# Autodesk Inventor assembly: S8x1
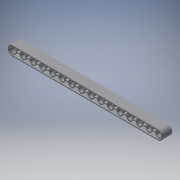
[picture p0: Inventor's stored thumbnail of the model, 180x180]
Saved by Autodesk Inventor 2019 (Build 230136000, 136)
## iProperties
Created: 2019-01-31
Part Number: S8x1
Document SubType Name: Assembly
Designer: Varga Daniel
Author: Varga Daniel
## Documents named in this file (3)
- C:\!_Dani\!_cloud\OneDrive\!_munka\Revolution\RevvyDemoKit\Structural parts\Straight Beams\S16x1.iam
- C:\!_Dani\!_cloud\OneDrive\!_munka\Revolution\RevvyDemoKit\Structural parts\Straight Beams\straight_beam_inner_part_single.ipt
- C:\!_Dani\!_cloud\OneDrive\!_munka\Revolution\RevvyDemoKit\Structural parts\Straight Beams\straight_beam_end_part_single.ipt
## Components (16 placed, 2 different names)
1. straight_beam_inner_part_single:1 — Mate:4, Mate:5, Flush:25, Flush:26, Flush:27, Flush:28, Flush:29, Flush:30
2. straight_beam_inner_part_single:2 — Mate:5, Flush:11, Flush:12, Mate:7, Flush:25, Flush:26
3. straight_beam_inner_part_single:3 — Mate:3, Mate:4, Flush:29, Flush:30
4. straight_beam_inner_part_single:4 — Mate:2, Mate:3, Flush:27, Flush:28, Flush:31, Flush:32
5. straight_beam_inner_part_single:5 — Mate:2, Flush:23, Flush:24, Flush:31, Flush:32, Mate:13
6. straight_beam_end_part_single:1 — Flush:41, Flush:42, Mate:18
7. straight_beam_end_part_single:2 — Flush:11, Flush:12, Mate:7
8. straight_beam_inner_part_single:6 — Flush:13, Flush:14, Mate:8, Flush:15, Flush:16, Mate:9
9. straight_beam_inner_part_single:7 — Flush:15, Flush:16, Mate:9, Flush:17, Flush:18, Mate:10
10. straight_beam_inner_part_single:8 — Flush:17, Flush:18, Mate:10, Flush:19, Flush:20, Mate:11
11. straight_beam_inner_part_single:9 — Flush:19, Flush:20, Mate:11, Flush:33, Flush:34, Mate:14
12. straight_beam_inner_part_single:10 — Flush:13, Flush:14, Mate:8, Flush:23, Flush:24, Mate:13
13. straight_beam_inner_part_single:11 — Flush:33, Flush:34, Flush:35, Flush:36, Mate:14, Mate:15
14. straight_beam_inner_part_single:12 — Flush:35, Flush:36, Flush:37, Flush:38, Mate:15, Mate:16
15. straight_beam_inner_part_single:13 — Flush:37, Flush:38, Flush:39, Flush:40, Mate:16, Mate:17
16. straight_beam_inner_part_single:14 — Flush:39, Flush:40, Flush:41, Flush:42, Mate:17, Mate:18
## Relationships (45: Flush 30, Mate 15)
- Mate:2: straight_beam_inner_part_single:4 ↔ straight_beam_inner_part_single:5
- Mate:3: straight_beam_inner_part_single:3 ↔ straight_beam_inner_part_single:4
- Mate:4: straight_beam_inner_part_single:1 ↔ straight_beam_inner_part_single:3
- Mate:5: straight_beam_inner_part_single:1 ↔ straight_beam_inner_part_single:2
- Flush:11: straight_beam_inner_part_single:2 ↔ straight_beam_end_part_single:2
- Flush:12: straight_beam_inner_part_single:2 ↔ straight_beam_end_part_single:2
- Mate:7: straight_beam_inner_part_single:2 ↔ straight_beam_end_part_single:2
- Flush:13: straight_beam_inner_part_single:6 ↔ straight_beam_inner_part_single:10
- Flush:14: straight_beam_inner_part_single:6 ↔ straight_beam_inner_part_single:10
- Mate:8: straight_beam_inner_part_single:6 ↔ straight_beam_inner_part_single:10
- Flush:15: straight_beam_inner_part_single:6 ↔ straight_beam_inner_part_single:7
- Flush:16: straight_beam_inner_part_single:6 ↔ straight_beam_inner_part_single:7
- Mate:9: straight_beam_inner_part_single:6 ↔ straight_beam_inner_part_single:7
- Flush:17: straight_beam_inner_part_single:7 ↔ straight_beam_inner_part_single:8
- Flush:18: straight_beam_inner_part_single:7 ↔ straight_beam_inner_part_single:8
- Mate:10: straight_beam_inner_part_single:7 ↔ straight_beam_inner_part_single:8
- Flush:19: straight_beam_inner_part_single:8 ↔ straight_beam_inner_part_single:9
- Flush:20: straight_beam_inner_part_single:8 ↔ straight_beam_inner_part_single:9
- Mate:11: straight_beam_inner_part_single:8 ↔ straight_beam_inner_part_single:9
- Flush:23: straight_beam_inner_part_single:5 ↔ straight_beam_inner_part_single:10
- Flush:24: straight_beam_inner_part_single:5 ↔ straight_beam_inner_part_single:10
- Flush:25: straight_beam_inner_part_single:1 ↔ straight_beam_inner_part_single:2
- Flush:26: straight_beam_inner_part_single:1 ↔ straight_beam_inner_part_single:2
- Flush:27: straight_beam_inner_part_single:1 ↔ straight_beam_inner_part_single:4
- Flush:28: straight_beam_inner_part_single:1 ↔ straight_beam_inner_part_single:4
- Flush:29: straight_beam_inner_part_single:1 ↔ straight_beam_inner_part_single:3
- Flush:30: straight_beam_inner_part_single:1 ↔ straight_beam_inner_part_single:3
- Flush:31: straight_beam_inner_part_single:4 ↔ straight_beam_inner_part_single:5
- Flush:32: straight_beam_inner_part_single:4 ↔ straight_beam_inner_part_single:5
- Mate:13: straight_beam_inner_part_single:5 ↔ straight_beam_inner_part_single:10
- Flush:33: straight_beam_inner_part_single:9 ↔ straight_beam_inner_part_single:11
- Flush:34: straight_beam_inner_part_single:9 ↔ straight_beam_inner_part_single:11
- Flush:35: straight_beam_inner_part_single:11 ↔ straight_beam_inner_part_single:12
- Flush:36: straight_beam_inner_part_single:11 ↔ straight_beam_inner_part_single:12
- Flush:37: straight_beam_inner_part_single:12 ↔ straight_beam_inner_part_single:13
- Flush:38: straight_beam_inner_part_single:12 ↔ straight_beam_inner_part_single:13
- Flush:39: straight_beam_inner_part_single:13 ↔ straight_beam_inner_part_single:14
- Flush:40: straight_beam_inner_part_single:13 ↔ straight_beam_inner_part_single:14
- Flush:41: straight_beam_end_part_single:1 ↔ straight_beam_inner_part_single:14
- Flush:42: straight_beam_end_part_single:1 ↔ straight_beam_inner_part_single:14
- Mate:14: straight_beam_inner_part_single:9 ↔ straight_beam_inner_part_single:11
- Mate:15: straight_beam_inner_part_single:11 ↔ straight_beam_inner_part_single:12
- Mate:16: straight_beam_inner_part_single:12 ↔ straight_beam_inner_part_single:13
- Mate:17: straight_beam_inner_part_single:13 ↔ straight_beam_inner_part_single:14
- Mate:18: straight_beam_end_part_single:1 ↔ straight_beam_inner_part_single:14
